# Autodesk Inventor assembly: Ankle_MIR
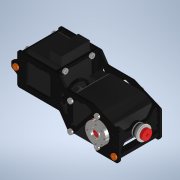
[picture p0: Inventor's stored thumbnail of the model, 180x180]
Saved by Autodesk Inventor 2020 (Build 240168000, 168)
## iProperties
Created: 2022-06-03
Part Number: Ankle_MIR
Document SubType Name: Assembly
Designer: Masato Kubotera
Author: Masato Kubotera
## Documents named in this file (17)
- C:\Users\MasatoKubotera\Documents\Inventor\SUSTAINA-OP\LowerBody\Ankle\Ankle_MIR.iam
- C:\Users\MasatoKubotera\Documents\Inventor\SUSTAINA-OP\LowerBody\Ankle\Ankle_side_frame.ipt
- C:\Users\MasatoKubotera\Documents\Inventor\SUSTAINA-OP\LowerBody\Ankle\Ankle_front_frame.ipt
- C:\Users\MasatoKubotera\Documents\Inventor\SUSTAINA-OP\LowerBody\Ankle\Ankle_back_frame.ipt
- C:\Users\MasatoKubotera\Documents\Inventor\SUSTAINA-OP\ReadyMade\KONDO\B3M-SC-1170-A_with_ClampHorn_AND_FreeHorn.iam
- C:\Users\MasatoKubotera\Documents\Inventor\SUSTAINA-OP\ReadyMade\KONDO\B3M-SC-1040-A_with_ClampHorn.iam
- C:\Users\MasatoKubotera\Documents\Inventor\SUSTAINA-OP\ReadyMade\Spacer\ABLSBF6-39.5-M3-N3.ipt
- C:\Users\MasatoKubotera\Documents\Inventor\SUSTAINA-OP\ReadyMade\InsertNut\S4-05-3W.ipt
- C:\Users\MasatoKubotera\Documents\Inventor\SUSTAINA-OP\ReadyMade\Washer\UUW-0412-10H.ipt
- C:\Users\MasatoKubotera\Documents\Inventor\SUSTAINA-OP\ReadyMade\Washer\CC-0612-15B.ipt
- C:\Users\MasatoKubotera\Documents\Inventor\SUSTAINA-OP\ReadyMade\Bush\80F-0603.ipt
- C:\Users\MasatoKubotera\Documents\Inventor\SUSTAINA-OP\ReadyMade\Washer\TT-0814-10.ipt
- C:\Users\MasatoKubotera\Documents\Inventor\SUSTAINA-OP\ReadyMade\Washer\UUW-0614-03H.ipt
- C:\Users\MasatoKubotera\Documents\Inventor\SUSTAINA-OP\ReadyMade\Screw\M3-6.ipt
- C:\Users\MasatoKubotera\Documents\Inventor\SUSTAINA-OP\ReadyMade\Screw\M2_6-15.ipt
- C:\Users\MasatoKubotera\Documents\Inventor\SUSTAINA-OP\ReadyMade\Screw\M2_6-20.ipt
- C:\Users\MasatoKubotera\Documents\Inventor\SUSTAINA-OP\ReadyMade\Screw\DBTS4-6-4-DHC.ipt
## Components (34 placed, 16 different names)
1. Ankle_side_frame:1 — フラッシュ:4, メイト:3, メイト:2, フラッシュ:5, メイト:5, メイト:4, 挿入:4, 挿入:3, 挿入:2, 挿入:1, 角度:1, 挿入:9, 角度:2, 挿入:11, 挿入:26, 挿入:28, 挿入:30, 挿入:31, 挿入:32, 挿入:33
2. Ankle_side_frame:2 — 挿入:12, 挿入:10, 挿入:8, 挿入:7, 挿入:6, 挿入:5, 挿入:27, 挿入:29, 挿入:34, 挿入:35, 挿入:42, 挿入:43
3. Ankle_front_frame:1 — フラッシュ:4, メイト:3, メイト:2, メイト:1, 挿入:19, 挿入:20
4. Ankle_back_frame:1 — 挿入:18, 挿入:17, 挿入:16, 挿入:15, 挿入:40, 挿入:41, 挿入:42, 挿入:43
5. Ankle_back_frame:2 — フラッシュ:5, メイト:5, メイト:4, 挿入:14, 挿入:13, 挿入:38, 挿入:39
6. B3M-SC-1170-A_with_ClampHorn_AND_FreeHorn:1 [sub-assembly] — 挿入:4, 挿入:3, 挿入:2, 挿入:1, フラッシュ:3, フラッシュ:2, フラッシュ:1, 挿入:8, 挿入:7, 挿入:6, 挿入:5
7. B3M-SC-1040-A_with_ClampHorn:1 [sub-assembly] — 挿入:18, 挿入:17, 挿入:16, 挿入:15, 挿入:14, 挿入:13
8. ABLSBF6-39.5-M3-N3:1 — 角度:1, 挿入:9, 挿入:10
9. ABLSBF6-39.5-M3-N3:2 — 角度:2, 挿入:11, 挿入:12
10. S4-05-3W:1 — メイト:1, 挿入:19
11. UUW-0412-10H:1 — 挿入:20, 挿入:21, 挿入:23
12. CC-0612-15B:1 — 挿入:21, 挿入:22
13. 80F-0603:1 — 挿入:22
14. TT-0814-10:1 — 挿入:25
15. UUW-0614-03H:1 — 挿入:25, 挿入:24
16. M3-6:1 — 挿入:26
17. M3-6:2 — 挿入:27
18. M3-6:3 — 挿入:28
19. M3-6:4 — 挿入:29
20. M2_6-15:1 — 挿入:30
21. M2_6-15:2 — 挿入:31
22. M2_6-15:3 — 挿入:32
23. M2_6-15:4 — 挿入:33
24. M2_6-20:1 — 挿入:34
25. M2_6-20:2 — 挿入:35
26. M2_6-20:3 — 挿入:38
27. M2_6-20:4 — 挿入:39
28. M2_6-15:5 — 挿入:40
29. M2_6-15:6 — 挿入:41
30. M2_6-15:7 — 挿入:42
31. M2_6-15:8 — 挿入:43
32. DBTS4-6-4-DHC:1 — 挿入:23, 挿入:24
33. M2_6-20:5 — 挿入:42
34. M2_6-20:6 — 挿入:43
## Relationships (55: Insert 43, Mate 6, Flush 4, Angle 2)
- フラッシュ:4 [Flush]: Ankle_side_frame:1 ↔ Ankle_front_frame:1
- メイト:3 [Mate] (0.025 mm): Ankle_side_frame:1 ↔ Ankle_front_frame:1
- メイト:2 [Mate] (0.025 mm): Ankle_side_frame:1 ↔ Ankle_front_frame:1
- フラッシュ:5 [Flush]: Ankle_side_frame:1 ↔ Ankle_back_frame:2
- メイト:5 [Mate] (0.025 mm): Ankle_side_frame:1 ↔ Ankle_back_frame:2
- メイト:4 [Mate] (0.025 mm): Ankle_side_frame:1 ↔ Ankle_back_frame:2
- 挿入:18 [Insert]: Ankle_back_frame:1 ↔ B3M-SC-1040-A_with_ClampHorn:1
- 挿入:17 [Insert]: Ankle_back_frame:1 ↔ B3M-SC-1040-A_with_ClampHorn:1
- 挿入:16 [Insert]: Ankle_back_frame:1 ↔ B3M-SC-1040-A_with_ClampHorn:1
- 挿入:15 [Insert]: Ankle_back_frame:1 ↔ B3M-SC-1040-A_with_ClampHorn:1
- 挿入:14 [Insert]: Ankle_back_frame:2 ↔ B3M-SC-1040-A_with_ClampHorn:1
- 挿入:13 [Insert]: Ankle_back_frame:2 ↔ B3M-SC-1040-A_with_ClampHorn:1
- 挿入:4 [Insert]: Ankle_side_frame:1 ↔ B3M-SC-1170-A_with_ClampHorn_AND_FreeHorn:1
- 挿入:3 [Insert]: Ankle_side_frame:1 ↔ B3M-SC-1170-A_with_ClampHorn_AND_FreeHorn:1
- 挿入:2 [Insert]: Ankle_side_frame:1 ↔ B3M-SC-1170-A_with_ClampHorn_AND_FreeHorn:1
- 挿入:1 [Insert]: Ankle_side_frame:1 ↔ B3M-SC-1170-A_with_ClampHorn_AND_FreeHorn:1
- フラッシュ:3 [Flush]: B3M-SC-1170-A_with_ClampHorn_AND_FreeHorn:1
- フラッシュ:2 [Flush]: B3M-SC-1170-A_with_ClampHorn_AND_FreeHorn:1
- フラッシュ:1 [Mate]: B3M-SC-1170-A_with_ClampHorn_AND_FreeHorn:1
- 角度:1 [Angle] (0 deg): Ankle_side_frame:1 ↔ ABLSBF6-39.5-M3-N3:1
- 挿入:9 [Insert]: Ankle_side_frame:1 ↔ ABLSBF6-39.5-M3-N3:1
- 角度:2 [Angle] (0 deg): Ankle_side_frame:1 ↔ ABLSBF6-39.5-M3-N3:2
- 挿入:11 [Insert]: Ankle_side_frame:1 ↔ ABLSBF6-39.5-M3-N3:2
- 挿入:12 [Insert]: Ankle_side_frame:2 ↔ ABLSBF6-39.5-M3-N3:2
- 挿入:10 [Insert]: Ankle_side_frame:2 ↔ ABLSBF6-39.5-M3-N3:1
- 挿入:8 [Insert]: Ankle_side_frame:2 ↔ B3M-SC-1170-A_with_ClampHorn_AND_FreeHorn:1
- 挿入:7 [Insert]: Ankle_side_frame:2 ↔ B3M-SC-1170-A_with_ClampHorn_AND_FreeHorn:1
- 挿入:6 [Insert]: Ankle_side_frame:2 ↔ B3M-SC-1170-A_with_ClampHorn_AND_FreeHorn:1
- 挿入:5 [Insert]: Ankle_side_frame:2 ↔ B3M-SC-1170-A_with_ClampHorn_AND_FreeHorn:1
- メイト:1 [Mate]: Ankle_front_frame:1 ↔ S4-05-3W:1
- 挿入:19 [Insert]: Ankle_front_frame:1 ↔ S4-05-3W:1
- 挿入:20 [Insert]: Ankle_front_frame:1 ↔ UUW-0412-10H:1
- 挿入:21 [Insert]: UUW-0412-10H:1 ↔ CC-0612-15B:1
- 挿入:22 [Insert]: CC-0612-15B:1 ↔ 80F-0603:1
- 挿入:23 [Insert]: UUW-0412-10H:1 ↔ DBTS4-6-4-DHC:1
- 挿入:26 [Insert]: Ankle_side_frame:1 ↔ M3-6:1
- 挿入:27 [Insert]: Ankle_side_frame:2 ↔ M3-6:2
- 挿入:28 [Insert]: Ankle_side_frame:1 ↔ M3-6:3
- 挿入:29 [Insert]: Ankle_side_frame:2 ↔ M3-6:4
- 挿入:30 [Insert]: Ankle_side_frame:1 ↔ M2_6-15:1
- 挿入:31 [Insert]: Ankle_side_frame:1 ↔ M2_6-15:2
- 挿入:32 [Insert]: Ankle_side_frame:1 ↔ M2_6-15:3
- 挿入:33 [Insert]: Ankle_side_frame:1 ↔ M2_6-15:4
- 挿入:34 [Insert]: Ankle_side_frame:2 ↔ M2_6-20:1
- 挿入:35 [Insert]: Ankle_side_frame:2 ↔ M2_6-20:2
- 挿入:38 [Insert]: Ankle_back_frame:2 ↔ M2_6-20:3
- 挿入:39 [Insert]: Ankle_back_frame:2 ↔ M2_6-20:4
- 挿入:40 [Insert]: Ankle_back_frame:1 ↔ M2_6-15:5
- 挿入:41 [Insert]: Ankle_back_frame:1 ↔ M2_6-15:6
- 挿入:42 [Insert]: Ankle_back_frame:1 ↔ M2_6-15:7
- 挿入:43 [Insert]: Ankle_back_frame:1 ↔ M2_6-15:8
- 挿入:25 [Insert]: TT-0814-10:1 ↔ UUW-0614-03H:1
- 挿入:24 [Insert]: UUW-0614-03H:1 ↔ DBTS4-6-4-DHC:1
- 挿入:42 [Insert]: Ankle_side_frame:2 ↔ M2_6-20:5
- 挿入:43 [Insert]: Ankle_side_frame:2 ↔ M2_6-20:6
